# Autodesk Inventor assembly: Gate
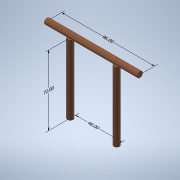
[picture p0: Inventor's stored thumbnail of the model, 180x180]
Saved by Autodesk Inventor 2020.1 (Build 241239000, 239)
## iProperties
Created: 2018-11-23
Part Number: Gate
Document SubType Name: Assembly
Designer: steele
Author: steele
## Documents named in this file (3)
- C:\git\CAD-Development\robSteele\HouseProjects\HorseGate\Gate.iam
- C:\git\CAD-Development\robSteele\HouseProjects\HorseGate\Post-6-Feet.ipt
- C:\git\CAD-Development\robSteele\HouseProjects\HorseGate\CrossMember-6-Feet.ipt
## Components (3 placed, 2 different names)
1. Post-6-Feet:1 — Insert:1
2. Post-6-Feet:2 — Insert:2
3. CrossMember-6-Feet:1 — Insert:1, Insert:2
## Relationships (2: Insert 2)
- Insert:1: Post-6-Feet:1 ↔ CrossMember-6-Feet:1
- Insert:2: Post-6-Feet:2 ↔ CrossMember-6-Feet:1
